# Autodesk Inventor assembly: Assembly2
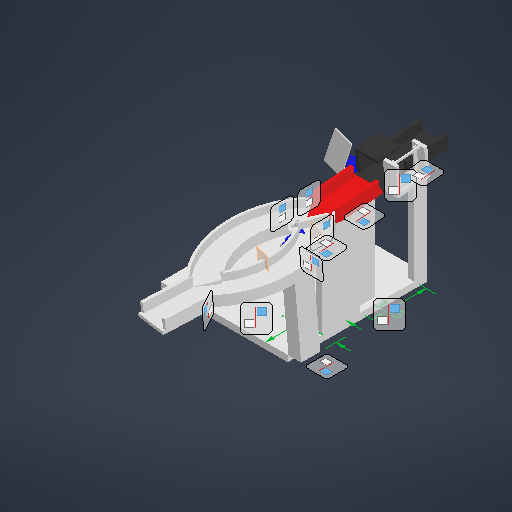
[picture p0: Inventor's stored thumbnail of the model, 512x512]
Saved by Autodesk Inventor 2026.2 (Build 302298000, 298)
## iProperties
Created: 2026-02-23
Part Number: Assembly2
Document SubType Name: Assembly
Designer: danda
Author: danda
## Documents named in this file (14)
- C:\Users\danda\BOM-project\Project\CAD\sorting\Assembly2.iam
- C:\Users\danda\BOM-project\Project\CAD\sorting\stand.ipt
- C:\Users\danda\BOM-project\Project\CAD\sorting\stand2.ipt
- C:\Users\danda\BOM-project\Project\CAD\sorting\inslide.ipt
- C:\Users\danda\BOM-project\Project\CAD\sorting\base.ipt
- C:\Users\danda\BOM-project\Project\CAD\sorting\Towerpro Micro Servo 9g\Towerpro Micro Servo 9g\Towerpro Micro Servo 9g.ipt
- C:\Users\danda\BOM-project\Project\CAD\sorting\motorstand1.ipt
- C:\Users\danda\BOM-project\Project\CAD\sorting\gate.ipt
- C:\Users\danda\BOM-project\Project\CAD\sorting\middleslide.ipt
- C:\Users\danda\BOM-project\Project\CAD\sorting\motorstand2.ipt
- C:\Users\danda\BOM-project\Project\CAD\sorting\gate2.ipt
- C:\Users\danda\BOM-project\Project\CAD\sorting\Sensorroom.ipt
- C:\Users\danda\BOM-project\Project\CAD\sorting\outside3.ipt
- C:\Users\danda\BOM-project\Project\CAD\sorting\outside32.ipt
## Components (15 placed, 13 different names)
1. stand:1 — Mate:5, Flush:8, Flush:9, Mate:30, Mate:33, Flush:14, Mate:34
2. stand2:1 — Mate:4, Flush:1, Flush:7, Mate:17, Mate:18, Mate:30, Mate:31, Mate:32, Flush:13
3. inslide:1 — Flush:8, Mate:17, Mate:18, Mate:31, Mate:32, Flush:13, Flush:18, Mate:42, Flush:20, Flush:21
4. base:1 — Mate:3, Mate:4, Flush:1, Mate:5, Mate:9, Mate:14, Mate:15, Flush:7, Flush:12, Flush:15, Mate:39, Mate:40, Mate:41
5. Towerpro Micro Servo 9g:1 — Mate:11, Mate:12, Mate:13, Insert:1
6. motorstand1:1 — Mate:9, Mate:11, Mate:12, Mate:13, Flush:12, Flush:15
7. gate:1 — Insert:1
8. middleslide:1 — Flush:9, Mate:33, Flush:14, Mate:34, Mate:43, Mate:44, Mate:45, Mate:46
9. motorstand2:1 — Mate:21, Mate:22, Mate:23, Mate:39, Mate:40, Mate:41
10. Towerpro Micro Servo 9g:2 — Mate:21, Mate:22, Mate:23, Insert:2, Rotational:1
11. gate2:1 — Insert:2, Rotational:1
12. Sensorroom:1 — Flush:18, Mate:42, Flush:20, Flush:21
13. outside3:1 — Mate:43, Mate:44
14. outside32:1 — Mate:45, Mate:46, Mate:47, Flush:22
15. middleslide:2 — Mate:47, Flush:22
## Relationships (43: Mate 28, Flush 12, Insert 2, RevoluteJoint 1)
- Mate:3: base:1
- Mate:4: stand2:1 ↔ base:1
- Flush:1: stand2:1 ↔ base:1
- Mate:5: stand:1 ↔ base:1
- Mate:9: base:1 ↔ motorstand1:1
- Mate:11: Towerpro Micro Servo 9g:1 ↔ motorstand1:1
- Mate:12: Towerpro Micro Servo 9g:1 ↔ motorstand1:1
- Mate:13: Towerpro Micro Servo 9g:1 ↔ motorstand1:1
- Insert:1: Towerpro Micro Servo 9g:1 ↔ gate:1
- Mate:14: base:1
- Mate:15: base:1
- Flush:7: stand2:1 ↔ base:1
- Flush:8: stand:1 ↔ inslide:1
- Mate:17: stand2:1 ↔ inslide:1
- Mate:18: stand2:1 ↔ inslide:1
- Flush:9: stand:1 ↔ middleslide:1
- Mate:21: motorstand2:1 ↔ Towerpro Micro Servo 9g:2
- Mate:22: motorstand2:1 ↔ Towerpro Micro Servo 9g:2
- Mate:23: motorstand2:1 ↔ Towerpro Micro Servo 9g:2
- Insert:2: Towerpro Micro Servo 9g:2 ↔ gate2:1
- Flush:12 (119.38 mm): base:1 ↔ motorstand1:1
- Mate:30 (85 mm): stand:1 ↔ stand2:1
- Mate:31: stand2:1 ↔ inslide:1
- Mate:32: stand2:1 ↔ inslide:1
- Flush:13: stand2:1 ↔ inslide:1
- Mate:33: stand:1 ↔ middleslide:1
- Flush:14: stand:1 ↔ middleslide:1
- Mate:34: stand:1 ↔ middleslide:1
- Flush:15 (10.16 mm): base:1 ↔ motorstand1:1
- Rotational:1 [RevoluteJoint]: Towerpro Micro Servo 9g:2 ↔ gate2:1
- Mate:39: base:1 ↔ motorstand2:1
- Mate:40: base:1 ↔ motorstand2:1
- Mate:41 (21.336 mm): base:1 ↔ motorstand2:1
- Flush:18: inslide:1 ↔ Sensorroom:1
- Mate:42: inslide:1 ↔ Sensorroom:1
- Flush:20: inslide:1 ↔ Sensorroom:1
- Flush:21: inslide:1 ↔ Sensorroom:1
- Mate:43: middleslide:1 ↔ outside3:1
- Mate:44: middleslide:1 ↔ outside3:1
- Mate:45: middleslide:1 ↔ outside32:1
- Mate:46: middleslide:1 ↔ outside32:1
- Mate:47: outside32:1 ↔ middleslide:2
- Flush:22: outside32:1 ↔ middleslide:2
## Named parameters: Finish2_Area = 90.88, Finish3_Area = 203.593, Finish4_Area = 203.593, Finish5_Area = 203.593
note: some values were not read from the file. Shown as the stored number, unit unknown: "Finish2_Area", "Finish3_Area", "Finish4_Area", "Finish5_Area".
